# Autodesk Inventor assembly: 43490-RadNabe
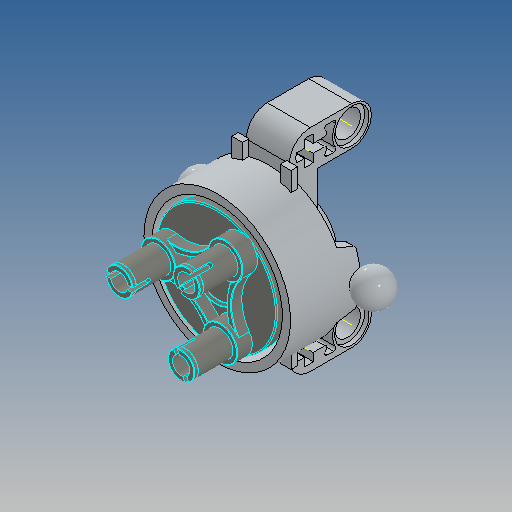
[picture p0: Inventor's stored thumbnail of the model, 512x512]
Saved by Autodesk Inventor 2025 (Build 290162010, 162A)
## iProperties
Created: 2024-11-18
Part Number: 43490-RadNabe
Material: Generisch
Document SubType Name: Assembly
Designer: hp.muther
Author: hp.muther
## Documents named in this file (3)
- D:\Inventor\Projekte\Muther\LEGO Technic\LEGO Pieces\43490-RadNabe.iam
- D:\Inventor\Projekte\Muther\LEGO Technic\LEGO Pieces\_Einzelteile zu Baugruppen\46490-darkstonegrey.ipt
- D:\Inventor\Projekte\Muther\LEGO Technic\LEGO Pieces\_Einzelteile zu Baugruppen\46490-interno.ipt
## Components (2 placed, 2 different names)
1. 46490-darkstonegrey:1 — Einfügen:1
2. 46490-interno:1 — Einfügen:1
## Relationships (1: Insert 1)
- Einfügen:1 [Insert] (-1.8 mm): 46490-darkstonegrey:1 ↔ 46490-interno:1
